# Autodesk Inventor assembly: ArmBackRight
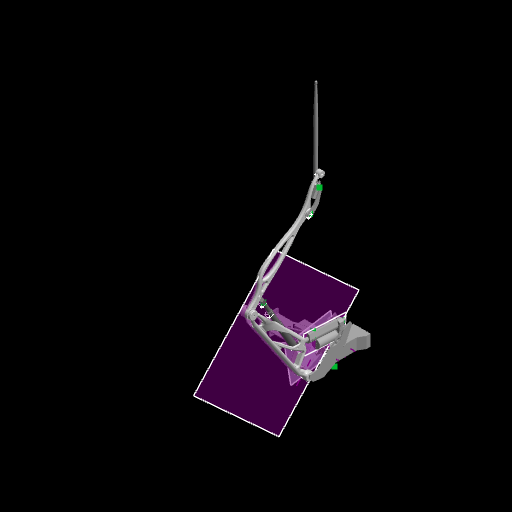
[picture p0: Inventor's stored thumbnail of the model, 512x512]
Saved by Autodesk Inventor 2025.2 (Build 292293000, 293)
## iProperties
Created: 2025-01-19
Part Number: ArmBackRight
Document SubType Name: Assembly
Designer: valer
Author: valer
## Documents named in this file (5)
- C:\Users\valer\Desktop\str1ker\cad\ArmBackRight.iam
- C:\Users\valer\Desktop\str1ker\cad\ArmBase.iam
- C:\Users\valer\Desktop\str1ker\cad\Arm.iam
- C:\Users\valer\Desktop\str1ker\cad\ArmScapulaLong.ipt
- C:\Users\valer\Desktop\str1ker\cad\ArmScapulaLongMirror.ipt
## Components (4 placed, 4 different names)
1. Base:1 [sub-assembly] — Mate:5, Mate:6, Mate:7, Mate:12, Mate:13, Mate:14, Mate:15, Mate:16, Mate:17
2. Arm:1 [sub-assembly] — Mate:5, Mate:6, Mate:8
3. ArmScapulaLong:2 — Mate:12, Mate:13, Mate:14
4. ArmScapulaLongMirror:1 — Mate:15, Mate:16, Mate:17
## Relationships (10: Mate 10)
- Mate:5: Base:1 ↔ Arm:1
- Mate:6: Base:1 ↔ Arm:1
- Mate:7: Base:1
- Mate:8: Arm:1
- Mate:12: Base:1 ↔ ArmScapulaLong:2
- Mate:13: Base:1 ↔ ArmScapulaLong:2
- Mate:14: Base:1 ↔ ArmScapulaLong:2
- Mate:15: Base:1 ↔ ArmScapulaLongMirror:1
- Mate:16: Base:1 ↔ ArmScapulaLongMirror:1
- Mate:17: Base:1 ↔ ArmScapulaLongMirror:1
